# Autodesk Inventor assembly: IV-6 Clock
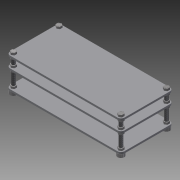
[picture p0: Inventor's stored thumbnail of the model, 180x180]
Saved by Autodesk Inventor 2015 (Build 190159000, 159)
## iProperties
Created: 2018-03-01
Part Number: IV-6 Clock
Document SubType Name: Assembly
Designer: Silas
Author: Silas
## Documents named in this file (6)
- D:\Skole\Viborg Tekniske Gymnasium - 3.G\Teknikfag\Eksamensprojekt\IV-6 Clock.iam
- D:\Skole\Viborg Tekniske Gymnasium - 3.G\Teknikfag\Eksamensprojekt\PCB1.ipt
- D:\Skole\Viborg Tekniske Gymnasium - 3.G\Teknikfag\Eksamensprojekt\PCB2.ipt
- D:\Skole\Viborg Tekniske Gymnasium - 3.G\Teknikfag\Eksamensprojekt\PCB3.ipt
- D:\Skole\Viborg Tekniske Gymnasium - 3.G\Teknikfag\Eksamensprojekt\AdjBolt.ipt
- D:\Skole\Viborg Tekniske Gymnasium - 3.G\Teknikfag\Eksamensprojekt\3MNut.ipt
## Components (27 placed, 5 different names)
1. PCB1:1 — Insert:1, Insert:2, Insert:3, Insert:4, Mate:5, Insert:21, Insert:22, Insert:23, Insert:24
2. PCB2:1 — Mate:1, Mate:2, Mate:5, Mate:6, Insert:13, Insert:14, Insert:15, Insert:16, Insert:17, Insert:18, Insert:19, Insert:20
3. PCB3:1 — Mate:3, Mate:4, Mate:6, Insert:5, Insert:6, Insert:7, Insert:8, Insert:9, Insert:10, Insert:11, Insert:12
4. AdjBolt:1 — Insert:1, Mate:1, Mate:4
5. AdjBolt:2 — Insert:2
6. AdjBolt:3 — Insert:3, Mate:2, Mate:3
7. AdjBolt:4 — Insert:4
8. 3MNut:1 — Insert:7
9. 3MNut:2 — Insert:8
10. 3MNut:3 — Insert:6
11. 3MNut:4 — Insert:5
12. 3MNut:5 — Insert:9
13. 3MNut:6 — Insert:10
14. 3MNut:7 — Insert:11
15. 3MNut:8 — Insert:12
16. 3MNut:9 — Insert:13
17. 3MNut:10 — Insert:14
18. 3MNut:11 — Insert:15
19. 3MNut:12 — Insert:16
20. 3MNut:13 — Insert:17
21. 3MNut:14 — Insert:18
22. 3MNut:15 — Insert:20
23. 3MNut:16 — Insert:19
24. 3MNut:17 — Insert:21
25. 3MNut:18 — Insert:22
26. 3MNut:19 — Insert:23
27. 3MNut:20 — Insert:24
## Relationships (30: Insert 24, Mate 6)
- Insert:1: PCB1:1 ↔ AdjBolt:1
- Insert:2: PCB1:1 ↔ AdjBolt:2
- Insert:3: PCB1:1 ↔ AdjBolt:3
- Insert:4: PCB1:1 ↔ AdjBolt:4
- Mate:1: PCB2:1 ↔ AdjBolt:1
- Mate:2: PCB2:1 ↔ AdjBolt:3
- Mate:3: PCB3:1 ↔ AdjBolt:3
- Mate:4: PCB3:1 ↔ AdjBolt:1
- Mate:5 (14 mm): PCB1:1 ↔ PCB2:1
- Mate:6 (8 mm): PCB2:1 ↔ PCB3:1
- Insert:5: PCB3:1 ↔ 3MNut:4
- Insert:6: PCB3:1 ↔ 3MNut:3
- Insert:7: PCB3:1 ↔ 3MNut:1
- Insert:8: PCB3:1 ↔ 3MNut:2
- Insert:9: PCB3:1 ↔ 3MNut:5
- Insert:10: PCB3:1 ↔ 3MNut:6
- Insert:11: PCB3:1 ↔ 3MNut:7
- Insert:12: PCB3:1 ↔ 3MNut:8
- Insert:13: PCB2:1 ↔ 3MNut:9
- Insert:14: PCB2:1 ↔ 3MNut:10
- Insert:15: PCB2:1 ↔ 3MNut:11
- Insert:16: PCB2:1 ↔ 3MNut:12
- Insert:17: PCB2:1 ↔ 3MNut:13
- Insert:18: PCB2:1 ↔ 3MNut:14
- Insert:19: PCB2:1 ↔ 3MNut:16
- Insert:20: PCB2:1 ↔ 3MNut:15
- Insert:21: PCB1:1 ↔ 3MNut:17
- Insert:22: PCB1:1 ↔ 3MNut:18
- Insert:23: PCB1:1 ↔ 3MNut:19
- Insert:24: PCB1:1 ↔ 3MNut:20
